# Autodesk Inventor assembly: robotassembly1
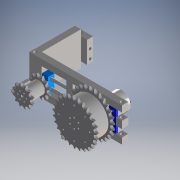
[picture p0: Inventor's stored thumbnail of the model, 180x180]
Saved by Autodesk Inventor 2016 (Build 200138000, 138)
## iProperties
Created: 2016-05-14
Part Number: robotassembly1
Document SubType Name: Assembly
Designer: hesaon
Author: hesaon
## Documents named in this file (14)
- C:\Users\Henrik Samuelsson\Documents\Killer-Bot-2016\AutodeskWorkspace\robotassembly1.iam
- C:\Users\Henrik Samuelsson\Documents\Killer-Bot-2016\AutodeskWorkspace\motorHolder57mmVer2.ipt
- C:\Users\Henrik Samuelsson\Documents\Killer-Bot-2016\AutodeskWorkspace\37D mm metal gearmotor.ipt
- C:\Users\Henrik Samuelsson\Documents\Killer-Bot-2016\AutodeskWorkspace\mountingHub6mm.ipt
- C:\Users\Henrik Samuelsson\Documents\Killer-Bot-2016\AutodeskWorkspace\sprocketsHolder.ipt
- C:\Users\Henrik Samuelsson\Documents\Killer-Bot-2016\AutodeskWorkspace\BigSprocket2.ipt
- C:\Users\Henrik Samuelsson\Documents\Killer-Bot-2016\AutodeskWorkspace\tracks_center.ipt
- C:\Users\Henrik Samuelsson\Documents\Killer-Bot-2016\AutodeskWorkspace\outerBigSprocket2.ipt
- C:\Users\Henrik Samuelsson\Documents\Killer-Bot-2016\AutodeskWorkspace\framesideRight.ipt
- C:\Users\Henrik Samuelsson\Documents\Killer-Bot-2016\AutodeskWorkspace\smallSprocketHolder.ipt
- C:\Users\Henrik Samuelsson\Documents\Killer-Bot-2016\AutodeskWorkspace\smallSprocket2.ipt
- C:\Users\Henrik Samuelsson\Documents\Killer-Bot-2016\AutodeskWorkspace\frameBack.ipt
- C:\Users\Henrik Samuelsson\Documents\Killer-Bot-2016\AutodeskWorkspace\pin5x60.ipt
- C:\Users\Henrik Samuelsson\Documents\Killer-Bot-2016\AutodeskWorkspace\smallSprocketFixture.ipt
## Components (16 placed, 12 different names)
1. motorHolder57mmVer2:1 — Insert:1, Insert:2, Insert:11, Insert:12
2. 37D mm metal gearmotor:1 — Insert:1, Insert:2, Insert:3
3. mountingHub6mm:1 — Insert:3, Insert:9, Insert:10
4. sprocketsHolder:2 — Insert:7, Insert:8, Mate:1, Mate:2, Mate:3, Mate:4
5. Roller Chain Sprocket1:2 — Insert:7, Insert:8
6. tracks_center:1
7. Outer big sprocket:1 — Mate:1, Mate:2, Mate:3, Mate:4, Insert:9, Insert:10
8. framesideRight:1 — Insert:11, Insert:12, Flush:1, Flush:2, Insert:19, Mate:5
9. smallSprocketHolder:1 — Insert:13, Insert:14, Insert:15, Insert:16
10. Roller Chain Sprocket1:3 — Insert:13, Insert:14
11. Roller Chain Sprocket1:4 — Insert:15, Insert:16, Insert:17, Insert:22
12. tracks_center:2 — Insert:17
13. frameBack:1 — Flush:1, Flush:2, Insert:18, Insert:20, Insert:21, Mate:5
14. pin5x60:1 — Insert:19
15. pin5x60:2 — Insert:18
16. smallSprocketFixture:1 — Insert:20, Insert:21, Insert:22
## Relationships (26: Insert 19, Mate 5, Flush 2)
- Insert:1: motorHolder57mmVer2:1 ↔ 37D mm metal gearmotor:1
- Insert:2: motorHolder57mmVer2:1 ↔ 37D mm metal gearmotor:1
- Insert:3: 37D mm metal gearmotor:1 ↔ mountingHub6mm:1
- Insert:7: sprocketsHolder:2 ↔ Roller Chain Sprocket1:2
- Insert:8: sprocketsHolder:2 ↔ Roller Chain Sprocket1:2
- Mate:1: sprocketsHolder:2 ↔ Outer big sprocket:1
- Mate:2: sprocketsHolder:2 ↔ Outer big sprocket:1
- Mate:3: sprocketsHolder:2 ↔ Outer big sprocket:1
- Mate:4: sprocketsHolder:2 ↔ Outer big sprocket:1
- Insert:9: mountingHub6mm:1 ↔ Outer big sprocket:1
- Insert:10: mountingHub6mm:1 ↔ Outer big sprocket:1
- Insert:11: motorHolder57mmVer2:1 ↔ framesideRight:1
- Insert:12: motorHolder57mmVer2:1 ↔ framesideRight:1
- Insert:13: smallSprocketHolder:1 ↔ Roller Chain Sprocket1:3
- Insert:14: smallSprocketHolder:1 ↔ Roller Chain Sprocket1:3
- Insert:15: smallSprocketHolder:1 ↔ Roller Chain Sprocket1:4
- Insert:16: smallSprocketHolder:1 ↔ Roller Chain Sprocket1:4
- Insert:17: Roller Chain Sprocket1:4 ↔ tracks_center:2
- Flush:1: framesideRight:1 ↔ frameBack:1
- Flush:2: framesideRight:1 ↔ frameBack:1
- Insert:18: frameBack:1 ↔ pin5x60:2
- Insert:19: framesideRight:1 ↔ pin5x60:1
- Insert:20: frameBack:1 ↔ smallSprocketFixture:1
- Insert:21: frameBack:1 ↔ smallSprocketFixture:1
- Mate:5: framesideRight:1 ↔ frameBack:1
- Insert:22 (6.5 mm): Roller Chain Sprocket1:4 ↔ smallSprocketFixture:1
